# Autodesk Inventor assembly: HBLFSNF5-SSU
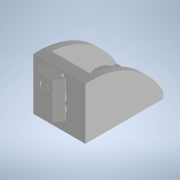
[picture p0: Inventor's stored thumbnail of the model, 180x180]
Saved by Autodesk Inventor 2021 (Build 250183000, 183)
## iProperties
Category: PARTsolutions
Company: MISUMI
Created: 2025-07-10
Part Number: HBLFSNF5-SSU
Catalog Web Link: www.cadenas.de
Description: HBLFSNF5-Tabbed Brackets - 1 Slots - HFS5 Series (Aluminum Extrusions 20, 25, 40 Square) - Reversal Tabbed Brackets (Depth 20mm)
Vendor: MISUMI
Document SubType Name: Assembly
Designer: psAdmin
Manufacturer: MISUMI
Mass: 6.77052 g
Surface Area: 53.2909 cm^2
Volume: 6.77052 cm^3
Density: 1 g/cm^3
Title: HBLFSNF5-SSU
Author: Cadenas PARTsolutions
Comments: Tabbed Brackets - 1 Slots - HFS5 Series (Aluminum Extrusions 20, 25, 40 Square) - Reversal Tabbed Brackets (Depth 20mm)
PSOL_IDENT_0: {$CADENAS_DATA/23d-libs/misumi/metric/38_al_extrusions_blackets/5/hblfsnf5_asmtab.prj},189 {VTYP=3D}
PSOL_IDENT_1: ,{STYP=ASSTAB},{NB=HBLFSNF5-SSU},{LINA=HBLFSNF5-SSU},{NN=HBLFSNF5},{DATE=16.09.2022 04:26:40},{GEOMD
PSOL_IDENT_2: ATE=29.08.2022 01:40:17},{VERSION=},{LINEID=10},{WBVAR=ALT1,ALT2},{WBNUMERIC=}  {NB=HBLFSNF5-SSU},{L
PSOL_IDENT_3: INA=HBLFSNF5-SSU},{KT=DUMMY},{PN=HBLFSNF5-SSU},{TYPE=HBLFSNF5},{AS=SCB5-10},{ASQ=2},{ATN=SHNTU5-5},{
PSOL_IDENT_4: ATNQ=2},{ALT1=},{ALT2=-SSU},{ALT2ALG= '' , 'w/o Applicable Screws and Nuts Set' , '-SET' , 'with SET
PSOL_IDENT_5: (Applicable Screws and Nuts Set)' , '-SST' , 'with SST (Applicable Screws and Nuts Set(Stainless St
PSOL_IDENT_6: eel))' , '-SEU' , 'with SEU (Applicable Screws and Nuts Set(Pre-Assembly Insertion Spring Nuts))' , '
PSOL_IDENT_7: -SSU' , 'with SSU (Applicable Screws and Nuts Set(Pre-Assembly Insertion Spring Nuts Stainless Steel
PSOL_IDENT_8: ))'  , '-SEP' , 'with SEP (Applicable Screws and Nuts Set(Post-Assembly Insertion Spring Nuts))' , '
PSOL_IDENT_9: -SSP' , 'with SSP (Applicable Screws and Nuts Set(Post-Assembly Insertion Spring Nuts Stainless Stee
PSOL_IDENT_10: l))', '-SEC' , 'with SEC (Applicable Screws and Nuts Set(Washer Integrated Screws and Nuts))' },{SMA
PSOL_IDENT_11: T=Sintering, 304 Stainless Steel Equivalent},{SALT2=2},{NALT2=2},{M=5},{PPATH=hblfsnf5/hblfsnf5_asmt
PSOL_IDENT_12: pl.prj}
NB: HBLFSNF5-SSU
NN: HBLFSNF5
NT: Tabbed Brackets - 1 Slots - HFS5 Series (Aluminum Extrusions 20, 25, 40 Square) - Reversal Tabbed Brackets (Depth 20mm)
NBSYN: $PN.
LINA: HBLFSNF5-SSU
CATALOG: Misumi
PN: HBLFSNF5-SSU
TYPE: HBLFSNF5
AS: SCB5-10
ASQ: 2
ATN: SHNTU5-5
ATNQ: 2
ALT1: w/o C (Mounting Holes for Cover)
ALT2: with SSU (Applicable Screws and Nuts Set(Pre-Assembly Insertion Spring Nuts Stainless Steel))
SUPPLIER: MISUMI
ARTICLENO: HBLFSNF5-SSU
BOMINFO: HBLFSNF5-SSU
CREATOR: CADENAS GmbH
## Documents named in this file (4)
- e:\temp\worker_COMMON_4\temp\tmp_1688_16_zKVSj\format_0\HBLFSNF5-SSU.iam
- e:\temp\worker_COMMON_4\temp\tmp_1688_16_zKVSj\format_0\HBLFSNF5-SSU_b.ipt
- e:\temp\worker_COMMON_4\temp\tmp_1688_16_zKVSj\format_0\SCB5-10.ipt
- e:\temp\worker_COMMON_4\temp\tmp_1688_16_zKVSj\format_0\SHNTU5-5.ipt
## Components (5 placed, 3 different names)
1. HBLFSNF5-SSU_b:1 — to_bolt1_XY@1 <-> bolt_XY@2, to_bolt1_Z@1 <-> bolt_Z@2, to_bolt1_YZ@1 <-> bolt_YZ@2, to_bolt2_XY@1 <-> bolt_XY@3, to_bolt2_Z@1 <-> bolt_Z@3, to_bolt2_YZ@1 <-> bolt_YZ@3, to_nut1_XY@1 <-> to_blackets_XY@4, to_nut1_Z@1 <-> to_blackets_Z@4, to_nut1_YZ@1 <-> to_blackets_YZ@4, to_nut2_XY@1 <-> to_blackets_XY@5, to_nut2_Z@1 <-> to_blackets_Z@5, to_nut2_YZ@1 <-> to_blackets_YZ@5
2. SCB5-10:1 — to_bolt1_XY@1 <-> bolt_XY@2, to_bolt1_Z@1 <-> bolt_Z@2, to_bolt1_YZ@1 <-> bolt_YZ@2
3. SCB5-10:2 — to_bolt2_XY@1 <-> bolt_XY@3, to_bolt2_Z@1 <-> bolt_Z@3, to_bolt2_YZ@1 <-> bolt_YZ@3
4. SHNTU5-5:1 — to_nut1_XY@1 <-> to_blackets_XY@4, to_nut1_Z@1 <-> to_blackets_Z@4, to_nut1_YZ@1 <-> to_blackets_YZ@4
5. SHNTU5-5:2 — to_nut2_XY@1 <-> to_blackets_XY@5, to_nut2_Z@1 <-> to_blackets_Z@5, to_nut2_YZ@1 <-> to_blackets_YZ@5
## Relationships (12: Mate 8, Angle 4)
- to_bolt1_XY@1 <-> bolt_XY@2 [Mate]: HBLFSNF5-SSU_b:1 ↔ SCB5-10:1
- to_bolt1_Z@1 <-> bolt_Z@2 [Mate]: HBLFSNF5-SSU_b:1 ↔ SCB5-10:1
- to_bolt1_YZ@1 <-> bolt_YZ@2 [Angle] (0 deg): HBLFSNF5-SSU_b:1 ↔ SCB5-10:1
- to_bolt2_XY@1 <-> bolt_XY@3 [Mate]: HBLFSNF5-SSU_b:1 ↔ SCB5-10:2
- to_bolt2_Z@1 <-> bolt_Z@3 [Mate]: HBLFSNF5-SSU_b:1 ↔ SCB5-10:2
- to_bolt2_YZ@1 <-> bolt_YZ@3 [Angle] (0 deg): HBLFSNF5-SSU_b:1 ↔ SCB5-10:2
- to_nut1_XY@1 <-> to_blackets_XY@4 [Mate]: HBLFSNF5-SSU_b:1 ↔ SHNTU5-5:1
- to_nut1_Z@1 <-> to_blackets_Z@4 [Mate]: HBLFSNF5-SSU_b:1 ↔ SHNTU5-5:1
- to_nut1_YZ@1 <-> to_blackets_YZ@4 [Angle] (0 deg): HBLFSNF5-SSU_b:1 ↔ SHNTU5-5:1
- to_nut2_XY@1 <-> to_blackets_XY@5 [Mate]: HBLFSNF5-SSU_b:1 ↔ SHNTU5-5:2
- to_nut2_Z@1 <-> to_blackets_Z@5 [Mate]: HBLFSNF5-SSU_b:1 ↔ SHNTU5-5:2
- to_nut2_YZ@1 <-> to_blackets_YZ@5 [Angle] (180 deg): HBLFSNF5-SSU_b:1 ↔ SHNTU5-5:2
